# Autodesk Inventor assembly: CIMple Box 1764
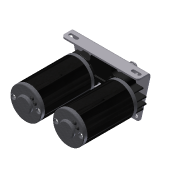
[picture p0: Inventor's stored thumbnail of the model, 180x180]
Saved by Autodesk Inventor 2011 (Build 150239000, 239)
## iProperties
Created: 2011-01-13
Part Number: CIMple Box 1764
Document SubType Name: Assembly
Designer: dfranz
Translation Standard: STEP AP203
FileName: S:/Products/Gearboxes Spur Single Stage/Single Stage Toughbox/CIMple Box.stp
PreProcessor: Unknown
PostProcessor: Build: 239, Release: 2011 RTM - Date: Wed 02/17/2010
Sent Units: millimeter
Uncertainty: 0.001
Author: dfranz
## Documents named in this file (16)
- R:\2010-2011\CMO\Web Site\CADalog\Motors\CIMple Box 1764.iam
- R:\CAD Archives\Motors\CIMple Box 1764\Single d03 1764.ipt
- R:\CAD Archives\Motors\CIMple Box 1764\Single d04 1764.ipt
- R:\CAD Archives\Motors\CIMple Box 1764\Single d02 1764.ipt
- R:\CAD Archives\Motors\CIMple Box 1764\Single d05 1764.ipt
- R:\CAD Archives\Motors\CIMple Box 1764\CIMple Box Sticker 1764.ipt
- R:\CAD Archives\Motors\CIMple Box 1764\Single d01 1764.ipt
- R:\CAD Archives\Motors\CIMple Box 1764\10-32x0625 SHCS 1764.ipt
- R:\CAD Archives\Motors\CIMple Box 1764\250 Washer 1764.ipt
- R:\CAD Archives\Motors\CIMple Box 1764\14-20x0500 BHCS 1764.ipt
- R:\CAD Archives\Motors\CIMple Box 1764\10-32 Nylock Nut 1764.ipt
- R:\CAD Archives\Motors\CIMple Box 1764\125x124x700 Key 1764.ipt
- R:\CAD Archives\Motors\CIMple Box 1764\8mm Spring Clip 1764.ipt
- R:\CAD Archives\Motors\CIMple Box 1764\R6ZZ 1764.ipt
- R:\CAD Archives\Motors\CIMple Box 1764\FR-8-ZZ 1764.ipt
- R:\CAD Archives\Motors\CIM Motor Dewalt Shifter 1764\CIM Motor 1764.ipt
## Components (28 placed, 15 different names)
1. Single d01 1764:1 — Mate:1, Mate:3, Mate:5, Mate:7
2. 10-32x0625 SHCS 1764:1 — Mate:6
3. 10-32x0625 SHCS 1764:2
4. 10-32x0625 SHCS 1764:3
5. 10-32x0625 SHCS 1764:4
6. 10-32x0625 SHCS 1764:5
7. 10-32x0625 SHCS 1764:6
8. 10-32x0625 SHCS 1764:7
9. 10-32x0625 SHCS 1764:8 — Mate:4
10. R6ZZ 1764:1
11. Single d03 1764:1
12. Single d04 1764:1
13. Single d02 1764:1
14. FR-8-ZZ 1764:1
15. 8mm Spring Clip 1764:1
16. 8mm Spring Clip 1764:2
17. 250 Washer 1764:1
18. 14-20x0500 BHCS 1764:1
19. Single d05 1764:1
20. Single d05 1764:2
21. CIMple Box Sticker 1764:1
22. 10-32 Nylock Nut 1764:1
23. 10-32 Nylock Nut 1764:2
24. 10-32 Nylock Nut 1764:3
25. 10-32 Nylock Nut 1764:4
26. 125x124x700 Key 1764:1
27. CIM Motor 1764:1 — Mate:1, Mate:6, Mate:7
28. CIM Motor 1764:2 — Mate:3, Mate:4, Mate:5
## Relationships (6: Mate 6)
- Mate:1: Single d01 1764:1 ↔ CIM Motor 1764:1
- Mate:3: Single d01 1764:1 ↔ CIM Motor 1764:2
- Mate:4: 10-32x0625 SHCS 1764:8 ↔ CIM Motor 1764:2
- Mate:5: Single d01 1764:1 ↔ CIM Motor 1764:2
- Mate:6: 10-32x0625 SHCS 1764:1 ↔ CIM Motor 1764:1
- Mate:7: Single d01 1764:1 ↔ CIM Motor 1764:1
